# Autodesk Inventor assembly: 00_XY_stage-CHUO_SEIKI_LD-647-R1
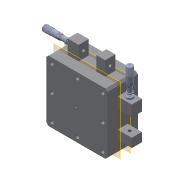
[picture p0: Inventor's stored thumbnail of the model, 180x180]
Saved by Autodesk Inventor 2019 (Build 230136000, 136)
## iProperties
Created: 2019-05-02
Part Number: 00_XY_stage-CHUO_SEIKI_LD-647-R1
Document SubType Name: Assembly
Designer: diederichbenedict
Author: diederichbenedict
## Documents named in this file (5)
- C:\Users\diederichbenedict\Dropbox\Dokumente\Promotion\PROJECTS\STORMoChip\INVENTOR\Nanoscopy-on-a-cheap\00_XY_stage-CHUO_SEIKI_LD-647-R1.iam
- C:\Users\diederichbenedict\Dropbox\Dokumente\Promotion\PROJECTS\STORMoChip\INVENTOR\Nanoscopy-on-a-cheap\00_XY_stage-CHUO_SEIKI_LD-647-R1-Top.ipt
- C:\Users\diederichbenedict\Dropbox\Dokumente\Promotion\PROJECTS\STORMoChip\INVENTOR\Nanoscopy-on-a-cheap\00_XY_stage-CHUO_SEIKI_LD-647-R1-Middle.ipt
- C:\Users\diederichbenedict\Dropbox\Dokumente\Promotion\PROJECTS\STORMoChip\INVENTOR\Nanoscopy-on-a-cheap\00_XY_stage-CHUO_SEIKI_LD-647-R1-Bottom.ipt
- C:\Users\diederichbenedict\Dropbox\Dokumente\Promotion\PROJECTS\STORMoChip\INVENTOR\Nanoscopy-on-a-cheap\00_XY_stage-CHUO_SEIKI_LD-647-R1-Micrometer.ipt
## Components (5 placed, 4 different names)
1. 00_XY_stage-CHUO_SEIKI_LD-647-R1-Top:1 — Flush:1, Flush:2, Mate:1
2. 00_XY_stage-CHUO_SEIKI_LD-647-R1-Middle:1 — Flush:1, Flush:2, Flush:3, Flush:4, Insert:1, Mate:1, Insert:2
3. 00_XY_stage-CHUO_SEIKI_LD-647-R1-Bottom:1 — Flush:3, Flush:4
4. 00_XY_stage-CHUO_SEIKI_LD-647-R1-Micrometer:1 — Insert:1
5. 00_XY_stage-CHUO_SEIKI_LD-647-R1-Micrometer:2 — Insert:2
## Relationships (7: Flush 4, Insert 2, Mate 1)
- Flush:1: 00_XY_stage-CHUO_SEIKI_LD-647-R1-Top:1 ↔ 00_XY_stage-CHUO_SEIKI_LD-647-R1-Middle:1
- Flush:2: 00_XY_stage-CHUO_SEIKI_LD-647-R1-Top:1 ↔ 00_XY_stage-CHUO_SEIKI_LD-647-R1-Middle:1
- Flush:3: 00_XY_stage-CHUO_SEIKI_LD-647-R1-Middle:1 ↔ 00_XY_stage-CHUO_SEIKI_LD-647-R1-Bottom:1
- Flush:4: 00_XY_stage-CHUO_SEIKI_LD-647-R1-Middle:1 ↔ 00_XY_stage-CHUO_SEIKI_LD-647-R1-Bottom:1
- Insert:1: 00_XY_stage-CHUO_SEIKI_LD-647-R1-Middle:1 ↔ 00_XY_stage-CHUO_SEIKI_LD-647-R1-Micrometer:1
- Mate:1: 00_XY_stage-CHUO_SEIKI_LD-647-R1-Top:1 ↔ 00_XY_stage-CHUO_SEIKI_LD-647-R1-Middle:1
- Insert:2: 00_XY_stage-CHUO_SEIKI_LD-647-R1-Middle:1 ↔ 00_XY_stage-CHUO_SEIKI_LD-647-R1-Micrometer:2
